# Autodesk Inventor assembly: Main Case Assembly
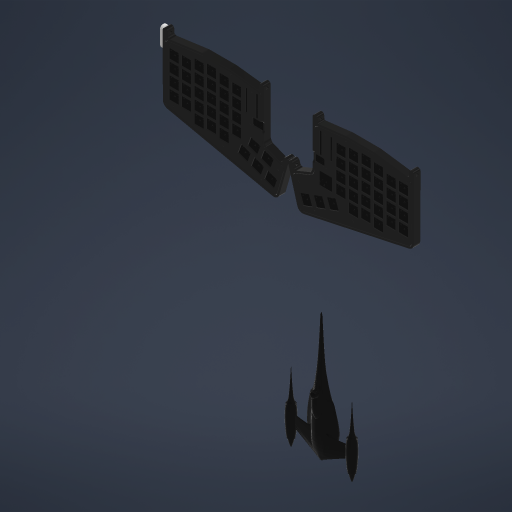
[picture p0: Inventor's stored thumbnail of the model, 512x512]
Saved by Autodesk Inventor 2024.3 (Build 283343000, 343)
## iProperties
Created: 2024-12-13
Part Number: Main Case Assembly
Document SubType Name: Assembly
Designer: micha
Author: micha
## Documents named in this file (8)
- C:\Users\micha\Documents\GitHub\clackenPersonal\Case Cad\Main Case Assembly.iam
- C:\Users\micha\Documents\GitHub\clackenPersonal\Case Cad\Split V2\Split V2\Split V2.ipt
- C:\Users\micha\Documents\GitHub\clackenPersonal\Case Cad\Case Bottom.ipt
- C:\Users\micha\Documents\GitHub\clackenPersonal\Case Cad\Top plate left.ipt
- C:\Users\micha\Documents\GitHub\clackenPersonal\Case Cad\Case Bottom_MIR1.ipt
- C:\Users\micha\Documents\GitHub\clackenPersonal\Case Cad\Top plate Right.ipt
- C:\Users\micha\Documents\GitHub\clackenPersonal\Case Cad\Stands.ipt
- C:\Users\micha\Downloads\AnyConv.com__N-1_Starfighter\N-1_Starfighter.ipt
## Components (8 placed, 7 different names)
1. Split V2:1 — Flush:1, Mate:1, Mate:2, Flush:3, Flush:4, Insert:3, Insert:4, Symmetry:1, Insert:7, Insert:8, Insert:13, Insert:14
2. Split V2:2 — Flush:1, Mate:1, Mate:2, Symmetry:1, Insert:11, Insert:12, Insert:15, Insert:16
3. Case Bottom:1 — Insert:13, Insert:14, Flush:5, Insert:17
4. Top plate left:1 — Flush:3, Flush:4, Insert:3, Insert:4, Insert:7, Insert:8
5. Case Bottom Right:1 — Insert:15, Insert:16
6. Top plate Right:1 — Insert:11, Insert:12
7. Stands:1 — Flush:5, Insert:17
8. N-1_Starfighter:1
## Relationships (18: Insert 11, Flush 4, Mate 2, Symmetry 1)
- Flush:1: Split V2:1 ↔ Split V2:2
- Mate:1 (76.2 mm): Split V2:1 ↔ Split V2:2
- Mate:2 (76.2 mm): Split V2:1 ↔ Split V2:2
- Flush:3: Split V2:1 ↔ Top plate left:1
- Flush:4: Split V2:1 ↔ Top plate left:1
- Insert:3: Split V2:1 ↔ Top plate left:1
- Insert:4: Split V2:1 ↔ Top plate left:1
- Symmetry:1: Split V2:1 ↔ Split V2:2
- Insert:7: Split V2:1 ↔ Top plate left:1
- Insert:8: Split V2:1 ↔ Top plate left:1
- Insert:11: Split V2:2 ↔ Top plate Right:1
- Insert:12: Split V2:2 ↔ Top plate Right:1
- Insert:13: Split V2:1 ↔ Case Bottom:1
- Insert:14: Split V2:1 ↔ Case Bottom:1
- Insert:15: Split V2:2 ↔ Case Bottom Right:1
- Insert:16: Split V2:2 ↔ Case Bottom Right:1
- Flush:5: Case Bottom:1 ↔ Stands:1
- Insert:17: Case Bottom:1 ↔ Stands:1
